# Autodesk Inventor assembly: Y_Axes
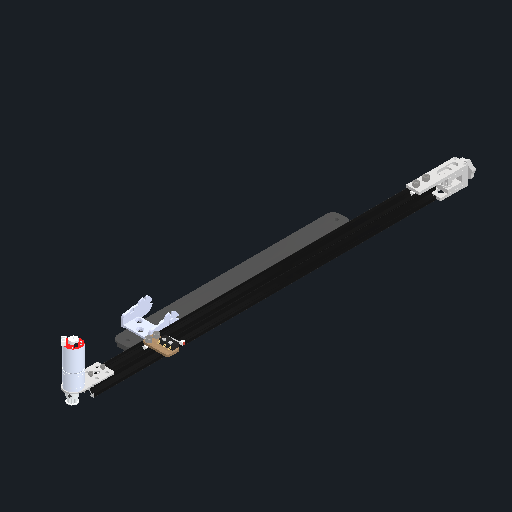
[picture p0: Inventor's stored thumbnail of the model, 512x512]
Saved by Autodesk Inventor 2027.1 (Build 311270010, 270A)
## iProperties
Created: 2026-10-02
Part Number: Y_Axes
Document SubType Name: Assembly
Designer: SDS Scholar
Author: SDS Scholar
## Documents named in this file (20)
- E:\Apps\AutodeskInventor\University\MCT333_Design_of_Mechatronics_Systems_1\CAD\cartesian_robot_workspace\Y_Axis.iam
- E:\Apps\AutodeskInventor\University\MCT333_Design_of_Mechatronics_Systems_1\CAD\off_the_shelf_components\AluminiumExtrusion\AluminiumExtrusion2020\Y_axis.ipt
- E:\Apps\AutodeskInventor\University\MCT333_Design_of_Mechatronics_Systems_1\CAD\off_the_shelf_components\GT2BeltTensioner\2020 Belt Tensioner G_K.ipt
- E:\Apps\AutodeskInventor\University\MCT333_Design_of_Mechatronics_Systems_1\CAD\off_the_shelf_components\T_nuts\Slider T-Nut for 2020 - M5.ipt
- C:\Users\SDS Scholar\Documents\Inventor\Content Center Files\R2027\en-US\SS-ISO 4762\ISO 4762 - M5 x 12SS-ISO.ipt
- E:\Apps\AutodeskInventor\University\MCT333_Design_of_Mechatronics_Systems_1\CAD\off_the_shelf_components\MotorMountPlate\motor holder bracket.ipt
- E:\Apps\AutodeskInventor\University\MCT333_Design_of_Mechatronics_Systems_1\CAD\off_the_shelf_components\T_nuts\Slider T-Nut for 2020 - M3.ipt
- C:\Users\SDS Scholar\Documents\Inventor\Content Center Files\R2027\en-US\ISO 4762(2)\ISO 4762 - M3 x 10ISO.ipt
- E:\Apps\AutodeskInventor\University\MCT333_Design_of_Mechatronics_Systems_1\CAD\cartesian_robot_workspace\LimitSwitchMountPlate.ipt
- C:\Users\SDS Scholar\Documents\Inventor\Content Center Files\R2027\en-US\SS-ISO 4762\ISO 4762 - M5 x 10SS-ISO.ipt
- E:\Apps\AutodeskInventor\University\MCT333_Design_of_Mechatronics_Systems_1\CAD\electronic_components\NO-NC Bump Switch\NO-NC Bump Switch.ipt
- C:\Users\SDS Scholar\Documents\Inventor\Content Center Files\R2027\en-US\DIN 7985 (H)\DIN 7985 (H) - M2.5x12-H.ipt
- C:\Users\SDS Scholar\Documents\Inventor\Content Center Files\R2027\en-US\ISO 4032(2)\ISO 4032 - M2.5 - ISO.ipt
- E:\Apps\AutodeskInventor\University\MCT333_Design_of_Mechatronics_Systems_1\CAD\motors_and_actuators\dc_motor_with_encoder\Motor\Motor.ipt
- C:\Users\SDS Scholar\Documents\Inventor\Content Center Files\R2027\en-US\ISO 7089\ISO 7089 - 3 - 140 HV(1).ipt
- C:\Users\SDS Scholar\Documents\Inventor\Content Center Files\R2027\en-US\ISO 7046-1 H(1)\ISO 7046-1 - M3 x 8_ - 4.8 - H - ISO.ipt
- E:\Apps\AutodeskInventor\University\MCT333_Design_of_Mechatronics_Systems_1\CAD\off_the_shelf_components\gt2_pulley_6\GT2 Pulley Assembly With Grub Screws\GT2 Pulley Assembly With Grub Screws.ipt
- E:\Apps\AutodeskInventor\University\MCT333_Design_of_Mechatronics_Systems_1\CAD\cartesian_robot_workspace\DragChainSupportMount.ipt
- E:\Apps\AutodeskInventor\University\MCT333_Design_of_Mechatronics_Systems_1\CAD\cartesian_robot_workspace\DragChainSupport.ipt
- E:\Apps\AutodeskInventor\University\MCT333_Design_of_Mechatronics_Systems_1\CAD\cartesian_robot_workspace\cable-chain-18x37\MountingHead\MountingHead.ipt
## Components (39 placed, 19 different names)
1. Y_axis:1 — Mate:1, Mate:2, Mate:3, Mate:4, Mate:5, Mate:6, Mate:7, Mate:10, Mate:13, Mate:14, Flush:1, Mate:15, Mate:16, Mate:17, Mate:18, Mate:21, Mate:22, Mate:25, Flush:2, Mate:26, Mate:27, Mate:28, Mate:36, Mate:39, Mate:42, Mate:57, Mate:72, Mate:73, Mate:74, Mate:75, Mate:76, Mate:77, Mate:78, Mate:79, Mate:86, Mate:87, Mate:88, Mate:93, Mate:94, Mate:95
2. MountingHead:1 — Mate:99, Mate:100, Angle:1
3. 2020 Belt Tensioner G_K:1 — Mate:8, Mate:11, Mate:14
4. SS ISO 4762 M5 x 12:1 — Mate:11, Mate:12, Mate:13
5. SS ISO 4762 M5 x 12:2 — Mate:8, Mate:9, Mate:10
6. Slider T-Nut for 2020 - M5:1 — Mate:4, Mate:5, Mate:9, Flush:1
7. Slider T-Nut for 2020 - M5:2 — Mate:6, Mate:7, Mate:12
8. motor holder bracket:1 — Mate:19, Mate:22, Mate:23, Mate:56, Mate:58, Mate:59, Mate:61, Mate:62, Mate:63, Mate:64, Mate:65, Mate:68
9. Slider T-Nut for 2020 - M3:1 — Mate:15, Mate:16, Mate:20
10. Slider T-Nut for 2020 - M3:2 — Mate:17, Mate:18, Mate:24, Flush:2
11. ISO 4762 M3 x 10:1 — Mate:23, Mate:24, Mate:25
12. ISO 4762 M3 x 10:2 — Mate:19, Mate:20, Mate:21
13. GT2 Pulley Assembly With Grub Screws:1 — Mate:70, Mate:71
14. Motor:1 — Mate:58, Mate:59, Mate:70
15. ISO 7089 3:1 — Mate:61, Mate:62, Mate:69
16. ISO 7089 3:2 — Mate:63, Mate:64, Mate:67
17. ISO 7046-1 H M3 x 8 - 4.8 - H:1 — Mate:67, Mate:68
18. ISO 7046-1 H M3 x 8 - 4.8 - H:2 — Mate:65, Mate:69, Mate:71
19. NO-NC Bump Switch:1 — Mate:45, Mate:47, Mate:48, Mate:49, Mate:51
20. LimitSwitchMountPlate:1 — Mate:36, Mate:37, Mate:40, Mate:46, Mate:48, Mate:50, Mate:54, Mate:55, Mate:56, Flush:100
21. Slider T-Nut for 2020 - M3:3 — Mate:28, Mate:41, Mate:57
22. Slider T-Nut for 2020 - M3:4 — Mate:26, Mate:27, Mate:38
23. SS ISO 4762 M5 x 10:1 — Mate:40, Mate:41, Mate:42
24. SS ISO 4762 M5 x 10:2 — Mate:37, Mate:38, Mate:39
25. DIN 7985 (H) M2.5x12-H:1 — Mate:45, Mate:46, Mate:47, Mate:52
26. DIN 7985 (H) M2.5x12-H:2 — Mate:49, Mate:50, Mate:51, Mate:53
27. ISO 4032 M2.5:1 — Mate:52, Mate:55
28. ISO 4032 M2.5:2 — Mate:53, Mate:54
29. DragChainSupportMount:1 — Mate:82, Mate:84, Mate:86, Mate:96, Flush:100
30. DragChainSupportMount:2 — Mate:89, Mate:91, Mate:93, Mate:97, Mate:98
31. Slider T-Nut for 2020 - M3:5 — Mate:78, Mate:79, Mate:92
32. Slider T-Nut for 2020 - M3:6 — Mate:76, Mate:77, Mate:90
33. Slider T-Nut for 2020 - M3:7 — Mate:72, Mate:73, Mate:85
34. Slider T-Nut for 2020 - M3:8 — Mate:74, Mate:75, Mate:83
35. ISO 4762 M3 x 10:3 — Mate:91, Mate:92, Mate:94
36. ISO 4762 M3 x 10:4 — Mate:84, Mate:85, Mate:88
37. ISO 4762 M3 x 10:5 — Mate:89, Mate:90, Mate:95
38. ISO 4762 M3 x 10:6 — Mate:82, Mate:83, Mate:87
39. DragChainSupport:1 — Mate:96, Mate:97, Mate:98, Mate:99, Mate:100, Angle:1
## Relationships (91: Mate 87, Flush 3, Angle 1)
- Mate:1: Y_axis:1
- Mate:2: Y_axis:1
- Mate:3: Y_axis:1
- Mate:4: Y_axis:1 ↔ Slider T-Nut for 2020 - M5:1
- Mate:5: Y_axis:1 ↔ Slider T-Nut for 2020 - M5:1
- Mate:6: Y_axis:1 ↔ Slider T-Nut for 2020 - M5:2
- Mate:7: Y_axis:1 ↔ Slider T-Nut for 2020 - M5:2
- Mate:8: 2020 Belt Tensioner G_K:1 ↔ SS ISO 4762 M5 x 12:2
- Mate:9: SS ISO 4762 M5 x 12:2 ↔ Slider T-Nut for 2020 - M5:1
- Mate:10: Y_axis:1 ↔ SS ISO 4762 M5 x 12:2
- Mate:11: 2020 Belt Tensioner G_K:1 ↔ SS ISO 4762 M5 x 12:1
- Mate:12: SS ISO 4762 M5 x 12:1 ↔ Slider T-Nut for 2020 - M5:2
- Mate:13: Y_axis:1 ↔ SS ISO 4762 M5 x 12:1
- Mate:14: Y_axis:1 ↔ 2020 Belt Tensioner G_K:1
- Flush:1: Y_axis:1 ↔ Slider T-Nut for 2020 - M5:1
- Mate:15: Y_axis:1 ↔ Slider T-Nut for 2020 - M3:1
- Mate:16: Y_axis:1 ↔ Slider T-Nut for 2020 - M3:1
- Mate:17: Y_axis:1 ↔ Slider T-Nut for 2020 - M3:2
- Mate:18: Y_axis:1 ↔ Slider T-Nut for 2020 - M3:2
- Mate:19: motor holder bracket:1 ↔ ISO 4762 M3 x 10:2
- Mate:20: Slider T-Nut for 2020 - M3:1 ↔ ISO 4762 M3 x 10:2
- Mate:21: Y_axis:1 ↔ ISO 4762 M3 x 10:2
- Mate:22: Y_axis:1 ↔ motor holder bracket:1
- Mate:23: motor holder bracket:1 ↔ ISO 4762 M3 x 10:1
- Mate:24: Slider T-Nut for 2020 - M3:2 ↔ ISO 4762 M3 x 10:1
- Mate:25: Y_axis:1 ↔ ISO 4762 M3 x 10:1
- Flush:2: Y_axis:1 ↔ Slider T-Nut for 2020 - M3:2
- Mate:26: Y_axis:1 ↔ Slider T-Nut for 2020 - M3:4
- Mate:27: Y_axis:1 ↔ Slider T-Nut for 2020 - M3:4
- Mate:28: Y_axis:1 ↔ Slider T-Nut for 2020 - M3:3
- Mate:36: Y_axis:1 ↔ LimitSwitchMountPlate:1
- Mate:37: LimitSwitchMountPlate:1 ↔ SS ISO 4762 M5 x 10:2
- Mate:38: Slider T-Nut for 2020 - M3:4 ↔ SS ISO 4762 M5 x 10:2
- Mate:39: Y_axis:1 ↔ SS ISO 4762 M5 x 10:2
- Mate:40: LimitSwitchMountPlate:1 ↔ SS ISO 4762 M5 x 10:1
- Mate:41: Slider T-Nut for 2020 - M3:3 ↔ SS ISO 4762 M5 x 10:1
- Mate:42: Y_axis:1 ↔ SS ISO 4762 M5 x 10:1
- Mate:45: NO-NC Bump Switch:1 ↔ DIN 7985 (H) M2.5x12-H:1
- Mate:46: LimitSwitchMountPlate:1 ↔ DIN 7985 (H) M2.5x12-H:1
- Mate:47: NO-NC Bump Switch:1 ↔ DIN 7985 (H) M2.5x12-H:1
- Mate:48: NO-NC Bump Switch:1 ↔ LimitSwitchMountPlate:1
- Mate:49: NO-NC Bump Switch:1 ↔ DIN 7985 (H) M2.5x12-H:2
- Mate:50: LimitSwitchMountPlate:1 ↔ DIN 7985 (H) M2.5x12-H:2
- Mate:51: NO-NC Bump Switch:1 ↔ DIN 7985 (H) M2.5x12-H:2
- Mate:52: DIN 7985 (H) M2.5x12-H:1 ↔ ISO 4032 M2.5:1
- Mate:53: DIN 7985 (H) M2.5x12-H:2 ↔ ISO 4032 M2.5:2
- Mate:54: LimitSwitchMountPlate:1 ↔ ISO 4032 M2.5:2
- Mate:55: LimitSwitchMountPlate:1 ↔ ISO 4032 M2.5:1
- Mate:56 (60 mm): motor holder bracket:1 ↔ LimitSwitchMountPlate:1
- Mate:57: Y_axis:1 ↔ Slider T-Nut for 2020 - M3:3
- Mate:58: motor holder bracket:1 ↔ Motor:1
- Mate:59: motor holder bracket:1 ↔ Motor:1
- Mate:61: motor holder bracket:1 ↔ ISO 7089 3:1
- Mate:62: motor holder bracket:1 ↔ ISO 7089 3:1
- Mate:63: motor holder bracket:1 ↔ ISO 7089 3:2
- Mate:64: motor holder bracket:1 ↔ ISO 7089 3:2
- Mate:65: motor holder bracket:1 ↔ ISO 7046-1 H M3 x 8 - 4.8 - H:2
- Mate:67: ISO 7089 3:2 ↔ ISO 7046-1 H M3 x 8 - 4.8 - H:1
- Mate:68: motor holder bracket:1 ↔ ISO 7046-1 H M3 x 8 - 4.8 - H:1
- Mate:69: ISO 7089 3:1 ↔ ISO 7046-1 H M3 x 8 - 4.8 - H:2
- Mate:70: GT2 Pulley Assembly With Grub Screws:1 ↔ Motor:1
- Mate:71: GT2 Pulley Assembly With Grub Screws:1 ↔ ISO 7046-1 H M3 x 8 - 4.8 - H:2
- Mate:72: Y_axis:1 ↔ Slider T-Nut for 2020 - M3:7
- Mate:73: Y_axis:1 ↔ Slider T-Nut for 2020 - M3:7
- Mate:74: Y_axis:1 ↔ Slider T-Nut for 2020 - M3:8
- Mate:75: Y_axis:1 ↔ Slider T-Nut for 2020 - M3:8
- Mate:76: Y_axis:1 ↔ Slider T-Nut for 2020 - M3:6
- Mate:77: Y_axis:1 ↔ Slider T-Nut for 2020 - M3:6
- Mate:78: Y_axis:1 ↔ Slider T-Nut for 2020 - M3:5
- Mate:79: Y_axis:1 ↔ Slider T-Nut for 2020 - M3:5
- Mate:82: DragChainSupportMount:1 ↔ ISO 4762 M3 x 10:6
- Mate:83: Slider T-Nut for 2020 - M3:8 ↔ ISO 4762 M3 x 10:6
- Mate:84: DragChainSupportMount:1 ↔ ISO 4762 M3 x 10:4
- Mate:85: Slider T-Nut for 2020 - M3:7 ↔ ISO 4762 M3 x 10:4
- Mate:86: Y_axis:1 ↔ DragChainSupportMount:1
- Mate:87: Y_axis:1 ↔ ISO 4762 M3 x 10:6
- Mate:88: Y_axis:1 ↔ ISO 4762 M3 x 10:4
- Mate:89: DragChainSupportMount:2 ↔ ISO 4762 M3 x 10:5
- Mate:90: Slider T-Nut for 2020 - M3:6 ↔ ISO 4762 M3 x 10:5
- Mate:91: DragChainSupportMount:2 ↔ ISO 4762 M3 x 10:3
- Mate:92: Slider T-Nut for 2020 - M3:5 ↔ ISO 4762 M3 x 10:3
- Mate:93: Y_axis:1 ↔ DragChainSupportMount:2
- Mate:94: Y_axis:1 ↔ ISO 4762 M3 x 10:3
- Mate:95: Y_axis:1 ↔ ISO 4762 M3 x 10:5
- Mate:96: DragChainSupportMount:1 ↔ DragChainSupport:1
- Mate:97: DragChainSupportMount:2 ↔ DragChainSupport:1
- Flush:100: LimitSwitchMountPlate:1 ↔ DragChainSupportMount:1
- Mate:98: DragChainSupportMount:2 ↔ DragChainSupport:1
- Mate:99: MountingHead:1 ↔ DragChainSupport:1
- Mate:100: MountingHead:1 ↔ DragChainSupport:1
- Angle:1 (0 deg): MountingHead:1 ↔ DragChainSupport:1
